# Autodesk Inventor assembly: 2020RobotV2
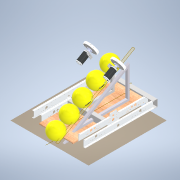
[picture p0: Inventor's stored thumbnail of the model, 180x180]
Saved by Autodesk Inventor 2020.2 (Build 242310000, 310)
## iProperties
Created: 2020-01-12
Part Number: 2020RobotV2
Document SubType Name: Assembly
Designer: robst
Author: robst
## Documents named in this file (13)
- C:\git\CAD-Development\robSteele\2020LongRobotBase\2020RobotV2.iam
- C:\git\CAD-Development\robSteele\2020LongRobotBase\2020 Wood Base.ipt
- C:\git\CAD-Development\robSteele\2020LongRobotBase\2020 End Plate.ipt
- C:\git\CAD-Development\robSteele\2020LongRobotBase\am-3921 AM14U4 Outside Plate.ipt
- C:\git\CAD-Development\robSteele\2020LongRobotBase\am-3922 AM14U4 Inside Plate.ipt
- C:\git\CAD-Development\robSteele\2020LongRobotBase\crossPlate.ipt
- C:\git\CAD-Development\robSteele\2020LongRobotBase\floor.ipt
- C:\git\CAD-Development\robSteele\2020LongRobotBase\ballSupport.ipt
- C:\git\CAD-Development\robSteele\2020LongRobotBase\ballSupport_MIR.ipt
- C:\git\CAD-Development\robSteele\2020LongRobotBase\1892-YEL.ipt
- C:\git\CAD-Development\robSteele\2020LongRobotBase\ceiling.ipt
- C:\git\CAD-Development\robSteele\2020LongRobotBase\shooter.iam
- C:\git\CAD-Development\robSteele\2020LongRobotBase\shooter_MIR.iam
## Components (18 placed, 12 different names)
1. 2020 Wood Base:1 — Flush:1, Mate:10, Mate:11, Mate:16, Mate:17, Flush:6, Mate:18, Flush:7, Mate:21, Mate:23
2. 2020 End Plate:1 — Flush:1, Mate:2, Mate:3, Mate:5, Mate:6, Flush:2, Flush:3, Mate:7, Mate:8, Mate:10, Mate:13, Mate:14
3. am-3921 AM14U4 Outside Plate:1 — Mate:5, Mate:6, Flush:2, Mate:15
4. am-3921 AM14U4 Outside Plate:2 — Mate:2, Mate:3, Flush:3, Mate:9
5. am-3922 AM14U4 Inside Plate:1 — Mate:7, Mate:8, Mate:9, Mate:11, Mate:12, Flush:4, Flush:5
6. crossPlate:1 — Mate:12, Flush:4, Flush:5
7. am-3922 AM14U4 Inside Plate:2 — Mate:13, Mate:14, Mate:15
8. floor:1 — Mate:16, Mate:17, Flush:6, Mate:19, Mate:25, Mate:27, Mate:29, Mate:30, Flush:8, Flush:9
9. ballSupport:1 — Mate:18, Mate:19, Flush:7, Mate:20, Mate:22, Mate:24, Mate:26, Mate:28
10. ballSupport_MIR:1
11. 1892-YEL:1 — Mate:20, Mate:21
12. 1892-YEL:2 — Mate:22, Mate:23
13. 1892-YEL:3 — Mate:24, Mate:25
14. 1892-YEL:4 — Mate:26, Mate:27
15. 1892-YEL:5 — Mate:28, Mate:29, Mate:31, Flush:10, Flush:11
16. ceiling:1 — Mate:30, Flush:8, Flush:9
17. shooter:1 [sub-assembly] — Mate:31, Flush:10, Flush:11
18. shooter_MIR:1 [sub-assembly]
## Relationships (40: Mate 29, Flush 11)
- Flush:1: 2020 Wood Base:1 ↔ 2020 End Plate:1
- Mate:2: 2020 End Plate:1 ↔ am-3921 AM14U4 Outside Plate:2
- Mate:3 (30.48 mm): 2020 End Plate:1 ↔ am-3921 AM14U4 Outside Plate:2
- Mate:5: 2020 End Plate:1 ↔ am-3921 AM14U4 Outside Plate:1
- Mate:6 (30.48 mm): 2020 End Plate:1 ↔ am-3921 AM14U4 Outside Plate:1
- Flush:2: 2020 End Plate:1 ↔ am-3921 AM14U4 Outside Plate:1
- Flush:3: 2020 End Plate:1 ↔ am-3921 AM14U4 Outside Plate:2
- Mate:7: 2020 End Plate:1 ↔ am-3922 AM14U4 Inside Plate:1
- Mate:8 (30.48 mm): 2020 End Plate:1 ↔ am-3922 AM14U4 Inside Plate:1
- Mate:9 (85.725 mm): am-3921 AM14U4 Outside Plate:2 ↔ am-3922 AM14U4 Inside Plate:1
- Mate:10: 2020 Wood Base:1 ↔ 2020 End Plate:1
- Mate:11: 2020 Wood Base:1 ↔ am-3922 AM14U4 Inside Plate:1
- Mate:12: am-3922 AM14U4 Inside Plate:1 ↔ crossPlate:1
- Flush:4: am-3922 AM14U4 Inside Plate:1 ↔ crossPlate:1
- Flush:5 (304.8 mm): am-3922 AM14U4 Inside Plate:1 ↔ crossPlate:1
- Mate:13: 2020 End Plate:1 ↔ am-3922 AM14U4 Inside Plate:2
- Mate:14: 2020 End Plate:1 ↔ am-3922 AM14U4 Inside Plate:2
- Mate:15 (85.725 mm): am-3921 AM14U4 Outside Plate:1 ↔ am-3922 AM14U4 Inside Plate:2
- Mate:16: 2020 Wood Base:1 ↔ floor:1
- Mate:17 (50.8 mm): 2020 Wood Base:1 ↔ floor:1
- Flush:6 (76.2 mm): 2020 Wood Base:1 ↔ floor:1
- Mate:18 (76.2 mm): 2020 Wood Base:1 ↔ ballSupport:1
- Mate:19: floor:1 ↔ ballSupport:1
- Flush:7: 2020 Wood Base:1 ↔ ballSupport:1
- Mate:20: ballSupport:1 ↔ 1892-YEL:1
- Mate:21: 2020 Wood Base:1 ↔ 1892-YEL:1
- Mate:22: ballSupport:1 ↔ 1892-YEL:2
- Mate:23: 2020 Wood Base:1 ↔ 1892-YEL:2
- Mate:24: ballSupport:1 ↔ 1892-YEL:3
- Mate:25: floor:1 ↔ 1892-YEL:3
- Mate:26: ballSupport:1 ↔ 1892-YEL:4
- Mate:27: floor:1 ↔ 1892-YEL:4
- Mate:28: ballSupport:1 ↔ 1892-YEL:5
- Mate:29: floor:1 ↔ 1892-YEL:5
- Mate:30 (711.2 mm): floor:1 ↔ ceiling:1
- Flush:8: floor:1 ↔ ceiling:1
- Flush:9: floor:1 ↔ ceiling:1
- Mate:31: 1892-YEL:5 ↔ shooter:1
- Flush:10: 1892-YEL:5 ↔ shooter:1
- Flush:11 (-127 mm): 1892-YEL:5 ↔ shooter:1
